# Autodesk Inventor assembly: V Wheel - Normal Spacer - Bolt v2
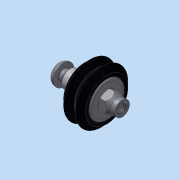
[picture p0: Inventor's stored thumbnail of the model, 180x180]
Saved by Autodesk Inventor 2013 (Build 170138000, 138)
## iProperties
Created: 2013-06-21
Part Number: V Wheel - Normal Spacer - Bolt v2
Document SubType Name: Assembly
Designer: Jon Hollander
Author: Jon Hollander
## Documents named in this file (5)
- D:\Dropbox\Research\CAD Library\v-slot\Part Assemblies\V Slot Wheel Assms\V Slot Wheel - Normal Spacer - Bolt\Workspaces\Workspace\PoC V2\Library Parts\VSlot Wheel SubAssms\V Wheel - Normal Spacer - Bolt v2.iam
- C:\Users\Work\Documents\Inventor\Content Center Files\R2013\en-US\Normal M5 Wheel Spacer\Normal M5 Wheel Spacer.ipt
- D:\Dropbox\Research\CAD Library\v-slot\V Wheel and Bearings.iam
- D:\Dropbox\Research\CAD Library\v-slot\Part Assemblies\Idler Pulley - Spacer - Bolt\Libraries\Content Center Files\en-US\ANSI B18.16.3M(2)\ANSI B18.16.3M - Property Class 5 and 10 - Metric M5 x 0.8 Top Insert Type.ipt
- D:\Dropbox\Research\CAD Library\v-slot\Part Assemblies\Idler Pulley - Spacer - Bolt\Libraries\Content Center Files\en-US\ANSI B18.3.4M(1)\ANSI B18.3.4M - M5 x 0.8 x 25(2).ipt
## Components (4 placed, 4 different names)
1. Broached Hexagon Socket Button Head Cap Screw - Metric M5 x 0.8 x 25:1 — Mate:12, Mate:14, Mate:15
2. Normal M5 Wheel Spacer Normal M5 Wheel Spacer:1 — Mate:14, Mate:16
3. V Wheel and Bearings:1 [sub-assembly] — Flush:1, Mate:15, Mate:16, Mate:17
4. Prevailing Torque Type Hex Nut - Steel Metric Property Class 5 and 10 - Metric M5 x 0.8 Top Insert Type:1 — Mate:12, Mate:17
## Relationships (7: Mate 6, Flush 1)
- [Mate]: Broached Hexagon Socket Button Head Cap Screw - Metric M5 x 0.8 x 25:1 ↔ Normal M5 Wheel Spacer Normal M5 Wheel Spacer:1
- Flush:1 (-0.5 mm): V Wheel and Bearings:1
- Mate:12: Broached Hexagon Socket Button Head Cap Screw - Metric M5 x 0.8 x 25:1 ↔ Prevailing Torque Type Hex Nut - Steel Metric Property Class 5 and 10 - Metric M5 x 0.8 Top Insert Type:1
- Mate:14 (3 mm): Broached Hexagon Socket Button Head Cap Screw - Metric M5 x 0.8 x 25:1 ↔ Normal M5 Wheel Spacer Normal M5 Wheel Spacer:1
- Mate:15: Broached Hexagon Socket Button Head Cap Screw - Metric M5 x 0.8 x 25:1 ↔ V Wheel and Bearings:1
- Mate:16: Normal M5 Wheel Spacer Normal M5 Wheel Spacer:1 ↔ V Wheel and Bearings:1
- Mate:17: V Wheel and Bearings:1 ↔ Prevailing Torque Type Hex Nut - Steel Metric Property Class 5 and 10 - Metric M5 x 0.8 Top Insert Type:1
